# Autodesk Inventor assembly: calf_left
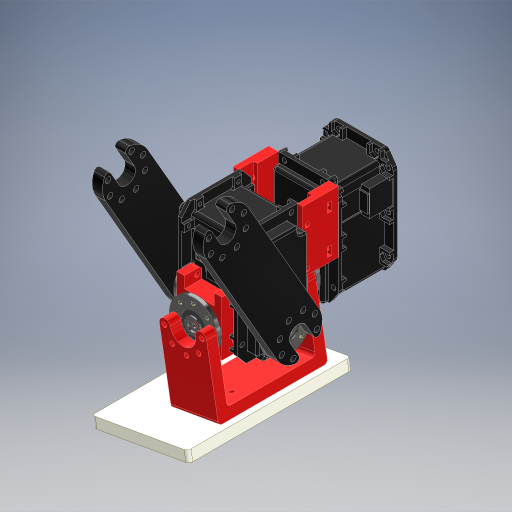
[picture p0: Inventor's stored thumbnail of the model, 512x512]
Saved by Autodesk Inventor 2024 (Build 280153000, 153)
## iProperties
Created: 2024-09-16
Part Number: calf_left
Document SubType Name: Assembly
Designer: msi
Author: msi
## Documents named in this file (13)
- C:\Users\msi\GITHUB\19th_intern_kgh_fight_robot\부품\Lower_Body\Calf\calf_right.iam
- C:\Users\msi\GITHUB\19th_intern_kgh_fight_robot\부품\Lower_Body\Calf\knee and ankle connection.ipt
- C:\Users\msi\GITHUB\19th_intern_kgh_fight_robot\부품\Lower_Body\Calf\ankle.ipt
- foot_right_64_ver2.ipt
- C:\Users\msi\GITHUB\19th_intern_kgh_fight_robot\부품\Lower_Body\Calf\behind ankle connection_outside.ipt
- C:\Users\msi\GITHUB\19th_intern_kgh_fight_robot\부품\Lower_Body\Calf\behind ankle connection_inside.ipt
- C:\Users\msi\GITHUB\19th_intern_kgh_fight_robot\부품\ROBOTIS(Inventor 2024 ver.)\다이나믹셀\MX-106T+idle.ipt.iam
- C:\Users\msi\GITHUB\19th_intern_kgh_fight_robot\부품\ROBOTIS(Inventor 2024 ver.)\다이나믹셀\MX-64T.ipt
- C:\Users\msi\GITHUB\19th_intern_kgh_fight_robot\부품\ROBOTIS(Inventor 2024 ver.)\혼\64-106Horn.ipt
- C:\Users\msi\GITHUB\19th_intern_kgh_fight_robot\부품\ROBOTIS(Inventor 2024 ver.)\아이들러\64아이들러.iam
- C:\Users\msi\GITHUB\19th_intern_kgh_fight_robot\부품\Lower_Body\Calf\foot.ipt
- C:\Users\msi\GITHUB\19th_intern_kgh_fight_robot\부품\Lower_Body\Calf\front ankle connection_right.ipt
- MX-106T+idle.ipt
## Components (12 placed, 10 different names)
1. behind ankle connection_outside:1 — 삽입:16, 삽입:17, 삽입:29, 삽입:30
2. behind ankle connection_inside:1 — 삽입:18, 삽입:19, 삽입:31
3. MX-64T:1 — 삽입:11, 삽입:16, 삽입:17, 삽입:18, 삽입:19
4. 64-106Horn:2 — 삽입:11, 삽입:24, 삽입:25
5. 64아이들러:1 [sub-assembly] — 삽입:28
6. foot:1 — 삽입:32, 삽입:33, 각도:2
7. knee and ankle connection:3 — 삽입:21, 플러쉬:1
8. MX-106T+idle.ipt:1 [sub-assembly] — 삽입:20, 삽입:21, 삽입:26, 삽입:27, 삽입:29, 삽입:30, 삽입:31, 각도:1, 각도:2
9. 64-106Horn:3 — 삽입:20, 삽입:22, 삽입:23
10. foot_right_64_ver2:1 — 삽입:24, 삽입:25, 삽입:32, 삽입:33
11. knee and ankle connection:4 — 삽입:22, 삽입:23, 각도:1, 플러쉬:1
12. front ankle connection_right:1 — 삽입:26, 삽입:27, 삽입:28
## Relationships (22: Insert 19, Angle 2, Flush 1)
- 삽입:11 [Insert]: MX-64T:1 ↔ 64-106Horn:2
- 삽입:16 [Insert]: behind ankle connection_outside:1 ↔ MX-64T:1
- 삽입:17 [Insert]: behind ankle connection_outside:1 ↔ MX-64T:1
- 삽입:18 [Insert]: behind ankle connection_inside:1 ↔ MX-64T:1
- 삽입:19 [Insert]: behind ankle connection_inside:1 ↔ MX-64T:1
- 삽입:20 [Insert]: MX-106T+idle.ipt:1 ↔ 64-106Horn:3
- 삽입:21 [Insert]: knee and ankle connection:3 ↔ MX-106T+idle.ipt:1
- 삽입:22 [Insert]: 64-106Horn:3 ↔ knee and ankle connection:4
- 삽입:23 [Insert]: 64-106Horn:3 ↔ knee and ankle connection:4
- 삽입:24 [Insert]: 64-106Horn:2 ↔ foot_right_64_ver2:1
- 삽입:25 [Insert]: 64-106Horn:2 ↔ foot_right_64_ver2:1
- 삽입:26 [Insert]: MX-106T+idle.ipt:1 ↔ front ankle connection_right:1
- 삽입:27 [Insert]: MX-106T+idle.ipt:1 ↔ front ankle connection_right:1
- 삽입:28 [Insert] (0.1 mm): 64아이들러:1 ↔ front ankle connection_right:1
- 삽입:29 [Insert]: behind ankle connection_outside:1 ↔ MX-106T+idle.ipt:1
- 삽입:30 [Insert]: behind ankle connection_outside:1 ↔ MX-106T+idle.ipt:1
- 삽입:31 [Insert]: behind ankle connection_inside:1 ↔ MX-106T+idle.ipt:1
- 삽입:32 [Insert]: foot:1 ↔ foot_right_64_ver2:1
- 삽입:33 [Insert]: foot:1 ↔ foot_right_64_ver2:1
- 각도:1 [Angle] (-30 deg): MX-106T+idle.ipt:1 ↔ knee and ankle connection:4
- 각도:2 [Angle] (190 deg): foot:1 ↔ MX-106T+idle.ipt:1
- 플러쉬:1 [Flush]: knee and ankle connection:3 ↔ knee and ankle connection:4
